# Autodesk Inventor assembly: assemby
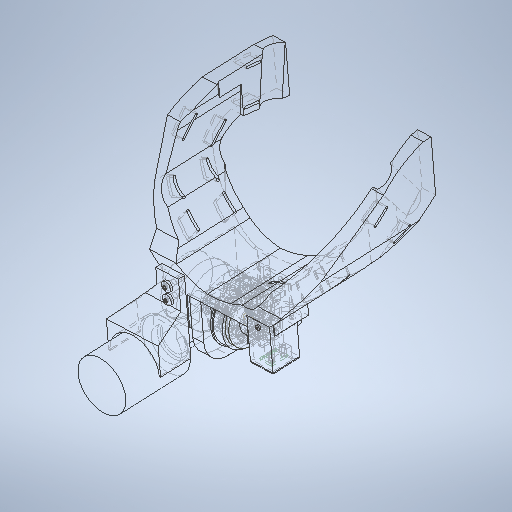
[picture p0: Inventor's stored thumbnail of the model, 512x512]
Saved by Autodesk Inventor 2025.2 (Build 292293000, 293)
## iProperties
Created: 2025-01-03
Part Number: assemby
Document SubType Name: Assembly
Designer: turbo
Author: turbo
## Documents named in this file (16)
- C:\Users\email\Desktop\Projects\Capstone\4TB6\CAD_Model\thigh_mount\thighmountassembly.iam
- C:\Users\email\Desktop\Projects\Capstone\4TB6\CAD_Model\thigh_mount\thighmount.ipt
- C:\Users\email\Desktop\Projects\Capstone\4TB6\CAD_Model\thigh_mount\motor.ipt
- C:\Users\email\Desktop\Projects\Capstone\4TB6\CAD_Model\thigh_mount\spool_temp.ipt
- C:\Users\email\Desktop\Projects\Capstone\4TB6\CAD_Model\thigh_mount\magnetholder.ipt
- C:\Users\email\Desktop\Projects\Capstone\4TB6\CAD_Model\thigh_mount\as5600mount.ipt
- C:\Users\email\Desktop\Projects\Capstone\4TB6\CAD_Model\thigh_mount\as5600.ipt
- C:\Users\email\Desktop\Projects\Capstone\4TB6\CAD_Model\thigh_mount\Lbracket.ipt
- C:\Users\email\Desktop\Projects\Capstone\4TB6\CAD_Model\thigh_mount\ANSI B18.6.7M - M6x1 x 10(6).ipt
- C:\Users\email\Desktop\Projects\Capstone\4TB6\CAD_Model\thigh_mount\motorsupport.ipt
- C:\Users\email\Desktop\Projects\Capstone\4TB6\CAD_Model\thigh_mount\ANSI B18.6.7M - M6x1 x 13(6).ipt
- C:\Users\email\Desktop\Projects\Capstone\4TB6\CAD_Model\thigh_mount\ANSI B18.6.7M - M6x1 x 16(6).ipt
- C:\Users\email\Desktop\Projects\Capstone\4TB6\CAD_Model\thigh_mount\IMU_temp.ipt
- C:\Users\email\Desktop\Projects\Capstone\4TB6\CAD_Model\thigh_mount\imu_mount.ipt
- C:\Users\email\Documents\Inventor\Content Center Files\R2025\en-US\ANSI B18.6.7M(02)\ANSI B18.6.7M - M3x0.5 x 10(6).ipt
- C:\Users\email\Desktop\Projects\Capstone\4TB6\CAD_Model\thigh_mount\pulleycase.ipt
## Components (21 placed, 15 different names)
1. thighmount:1 — Mate:1, Mate:15, Mate:16, Mate:17, Mate:18, Mate:25, Mate:26, Mate:27, Mate:36, Mate:38, Mate:40, Mate:42, Mate:43, Mate:44, Mate:45, Mate:46, Mate:47, Mate:48, Mate:49, Mate:50, Mate:51, Mate:62
2. motor:1 — Mate:15, Mate:16, Mate:17, Mate:18, Mate:19, Mate:20, Mate:21
3. spool_temp:1 — Mate:19, Mate:20, Mate:21, Mate:22, Mate:23, Mate:24
4. magnetholder:1 — Mate:22, Mate:23, Mate:24
5. as5600mount:1 — Mate:25, Mate:26, Mate:27, Mate:28, Mate:29, Mate:30
6. as5600:2 — Mate:28, Mate:29, Mate:30
7. Lbracket:1 — Mate:42, Mate:43, Insert:5
8. Lbracket:2 — Mate:44, Mate:45, Insert:6
9. Square Recessed Pan Head Machine Screw - Type III - Metric M6x1 x 10:1 — Mate:36, Mate:37, Mate:61
10. Square Recessed Pan Head Machine Screw - Type III - Metric M6x1 x 10:2 — Mate:38, Mate:39, Mate:59
11. Square Recessed Pan Head Machine Screw - Type III - Metric M6x1 x 10:3 — Mate:40, Mate:41, Mate:60
12. motorsupport:1 — Mate:46, Mate:47, Mate:48, Insert:7, Insert:8
13. Square Recessed Pan Head Machine Screw - Type III - Metric M6x1 x 13:1 — Insert:5
14. Square Recessed Pan Head Machine Screw - Type III - Metric M6x1 x 13:2 — Insert:6
15. Square Recessed Pan Head Machine Screw - Type III - Metric M6x1 x 16:1 — Insert:7
16. Square Recessed Pan Head Machine Screw - Type III - Metric M6x1 x 16:2 — Insert:8
17. imu_mount:1 — Mate:49, Mate:50, Mate:51, Mate:56, Mate:57, Mate:58
18. Square Recessed Pan Head Machine Screw - Type III - Metric M3x0.5 x 10:2
19. Square Recessed Pan Head Machine Screw - Type III - Metric M3x0.5 x 10:1
20. IMU_temp:1 — Mate:56, Mate:57, Mate:58
21. pulleycase:1 — Mate:59, Mate:60, Mate:61, Mate:62, Mate:37, Mate:41, Mate:39
## Relationships (48: Mate 44, Insert 4)
- Mate:1: thighmount:1
- Mate:15: thighmount:1 ↔ motor:1
- Mate:16: thighmount:1 ↔ motor:1
- Mate:17: thighmount:1 ↔ motor:1
- Mate:18: thighmount:1 ↔ motor:1
- Mate:19: motor:1 ↔ spool_temp:1
- Mate:20: motor:1 ↔ spool_temp:1
- Mate:21: motor:1 ↔ spool_temp:1
- Mate:22: spool_temp:1 ↔ magnetholder:1
- Mate:23: spool_temp:1 ↔ magnetholder:1
- Mate:24: spool_temp:1 ↔ magnetholder:1
- Mate:25: thighmount:1 ↔ as5600mount:1
- Mate:26: thighmount:1 ↔ as5600mount:1
- Mate:27: thighmount:1 ↔ as5600mount:1
- Mate:28: as5600mount:1 ↔ as5600:2
- Mate:29: as5600mount:1 ↔ as5600:2
- Mate:30: as5600mount:1 ↔ as5600:2
- Mate:36: thighmount:1 ↔ Square Recessed Pan Head Machine Screw - Type III - Metric M6x1 x 10:1
- Mate:37: Square Recessed Pan Head Machine Screw - Type III - Metric M6x1 x 10:1 ↔ pulleycase:1
- Mate:38: thighmount:1 ↔ Square Recessed Pan Head Machine Screw - Type III - Metric M6x1 x 10:2
- Mate:39: Square Recessed Pan Head Machine Screw - Type III - Metric M6x1 x 10:2 ↔ pulleycase:1
- Mate:40: thighmount:1 ↔ Square Recessed Pan Head Machine Screw - Type III - Metric M6x1 x 10:3
- Mate:41: Square Recessed Pan Head Machine Screw - Type III - Metric M6x1 x 10:3 ↔ pulleycase:1
- Mate:42: thighmount:1 ↔ Lbracket:1
- Mate:43: thighmount:1 ↔ Lbracket:1
- Mate:44: thighmount:1 ↔ Lbracket:2
- Mate:45: thighmount:1 ↔ Lbracket:2
- Mate:46: thighmount:1 ↔ motorsupport:1
- Mate:47: thighmount:1 ↔ motorsupport:1
- Mate:48: thighmount:1 ↔ motorsupport:1
- Insert:5: Lbracket:1 ↔ Square Recessed Pan Head Machine Screw - Type III - Metric M6x1 x 13:1
- Insert:6: Lbracket:2 ↔ Square Recessed Pan Head Machine Screw - Type III - Metric M6x1 x 13:2
- Insert:7: motorsupport:1 ↔ Square Recessed Pan Head Machine Screw - Type III - Metric M6x1 x 16:1
- Insert:8: motorsupport:1 ↔ Square Recessed Pan Head Machine Screw - Type III - Metric M6x1 x 16:2
- Mate:49: thighmount:1 ↔ imu_mount:1
- Mate:50 (0.25 mm): thighmount:1 ↔ imu_mount:1
- Mate:51: thighmount:1 ↔ imu_mount:1
- [Mate]: imu_mount:1 ↔ Square Recessed Pan Head Machine Screw - Type III - Metric M3x0.5 x 10:2
- [Mate]: imu_mount:1 ↔ Square Recessed Pan Head Machine Screw - Type III - Metric M3x0.5 x 10:2
- [Mate]: imu_mount:1 ↔ Square Recessed Pan Head Machine Screw - Type III - Metric M3x0.5 x 10:1
- [Mate]: imu_mount:1 ↔ Square Recessed Pan Head Machine Screw - Type III - Metric M3x0.5 x 10:1
- Mate:56: imu_mount:1 ↔ IMU_temp:1
- Mate:57: imu_mount:1 ↔ IMU_temp:1
- Mate:58: imu_mount:1 ↔ IMU_temp:1
- Mate:59: Square Recessed Pan Head Machine Screw - Type III - Metric M6x1 x 10:2 ↔ pulleycase:1
- Mate:60: Square Recessed Pan Head Machine Screw - Type III - Metric M6x1 x 10:3 ↔ pulleycase:1
- Mate:61: Square Recessed Pan Head Machine Screw - Type III - Metric M6x1 x 10:1 ↔ pulleycase:1
- Mate:62: thighmount:1 ↔ pulleycase:1
